# Autodesk Inventor assembly: emergency_stop
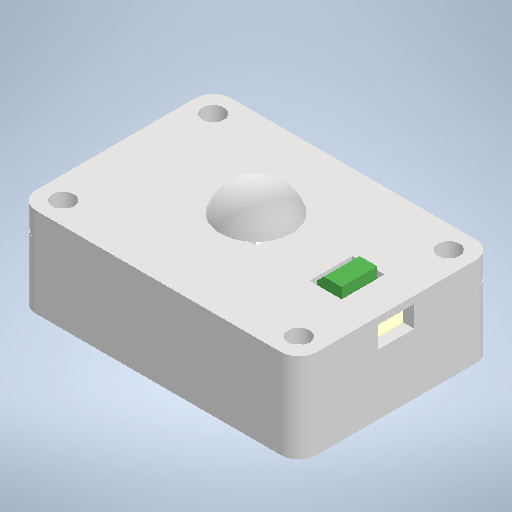
[picture p0: Inventor's stored thumbnail of the model, 512x512]
Saved by Autodesk Inventor 2025 (Build 290162000, 162)
## iProperties
Created: 2026-02-25
Part Number: emergency_stop
Document SubType Name: Assembly
Designer: sooo1
Author: sooo1
## Documents named in this file (7)
- C:\Users\sooo1\Documents\Inventor\MOBITOUCH\final\emergency_stop.iam
- C:\Users\sooo1\Documents\Inventor\MOBITOUCH\final\terminalblock.ipt
- C:\Users\sooo1\Documents\Inventor\MOBITOUCH\final\circuitboard.ipt
- C:\Users\sooo1\Documents\Inventor\MOBITOUCH\final\switch.ipt
- C:\Users\sooo1\Documents\Inventor\MOBITOUCH\final\enclosure.ipt
- C:\Users\sooo1\Documents\Inventor\MOBITOUCH\final\lid.ipt
- C:\Users\sooo1\Documents\Inventor\MOBITOUCH\final\nob_L.ipt
## Components (6 placed, 6 different names)
1. terminalblock:1 — フラッシュ:5, フラッシュ:6, フラッシュ:9
2. circuitboard:1 — フラッシュ:1, フラッシュ:2, フラッシュ:3, フラッシュ:4, フラッシュ:5, フラッシュ:6, フラッシュ:7, フラッシュ:10
3. switch:1 — フラッシュ:4, フラッシュ:7, フラッシュ:8, フラッシュ:9, フラッシュ:12
4. enclosure:1 — フラッシュ:10, フラッシュ:11
5. lid:1 — フラッシュ:11
6. nob_L:1 — フラッシュ:12
## Relationships (12: Flush 12)
- フラッシュ:1 [Flush]: circuitboard:1
- フラッシュ:2 [Flush]: circuitboard:1
- フラッシュ:3 [Flush]: circuitboard:1
- フラッシュ:4 [Flush]: circuitboard:1 ↔ switch:1
- フラッシュ:5 [Flush]: terminalblock:1 ↔ circuitboard:1
- フラッシュ:6 [Flush]: terminalblock:1 ↔ circuitboard:1
- フラッシュ:7 [Flush]: circuitboard:1 ↔ switch:1
- フラッシュ:8 [Flush]: switch:1
- フラッシュ:9 [Flush] (25 mm): terminalblock:1 ↔ switch:1
- フラッシュ:10 [Flush]: circuitboard:1 ↔ enclosure:1
- フラッシュ:11 [Flush]: enclosure:1 ↔ lid:1
- フラッシュ:12 [Flush]: switch:1 ↔ nob_L:1
